# Autodesk Inventor assembly: PBLMK-041-A
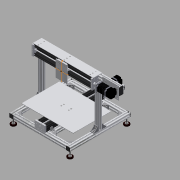
[picture p0: Inventor's stored thumbnail of the model, 180x180]
Saved by Autodesk Inventor 2016 (Build 200138000, 138)
## iProperties
Created: 2023-12-03
Part Number: PBLMK-041-A
Document SubType Name: Assembly
Designer: Riskinova Oktavia
Checked By: RIDWAN
Engr Approved By: RIDWAN
Company: POLITEKNIK NEGERI BATAM
Author: Riskinova Oktavia
Title: MINI CNC ENGRAVER
## Documents named in this file (56)
- D:\PROJECT NOVA 2021-2022\PBLMK-041\NEW KONSEP\PBLMK-041-A.iam
- D:\PROJECT NOVA 2021-2022\PBLMK-041\NEW KONSEP\SKETCH.ipt
- D:\PROJECT NOVA 2021-2022\PBLMK-041\NEW KONSEP\PBLMK-041-A\Frame\Frame0001.iam
- D:\PROJECT NOVA 2021-2022\PBLMK-041\NEW KONSEP\LINEAR ACTUATOR.iam
- D:\PROJECT NOVA 2021-2022\PBLMK-041\PBLMK-041\Solid33.ipt
- D:\PROJECT NOVA 2021-2022\PBLMK-041\PBLMK-041\Solid45.ipt
- D:\PROJECT NOVA 2021-2022\PBLMK-041\PBLMK-041\Solid39.ipt
- D:\PROJECT NOVA 2021-2022\PBLMK-041\PBLMK-041\Solid41.ipt
- D:\PROJECT NOVA 2021-2022\PBLMK-041\PBLMK-041\Solid43.ipt
- D:\PROJECT NOVA 2021-2022\PBLMK-041\PBLMK-041\Solid44.ipt
- D:\PROJECT NOVA 2021-2022\PBLMK-041\PBLMK-041\Solid57.ipt
- D:\PROJECT NOVA 2021-2022\PBLMK-041\PBLMK-041\Solid58.ipt
- D:\PROJECT NOVA 2021-2022\PBLMK-041\PBLMK-041\Solid31.ipt
- D:\PROJECT NOVA 2021-2022\PBLMK-041\PBLMK-041\Solid32.ipt
- D:\PROJECT NOVA 2021-2022\PBLMK-041\PBLMK-041\Solid1.ipt
- D:\PROJECT NOVA 2021-2022\PBLMK-041\PBLMK-041\Solid53.ipt
- D:\PROJECT NOVA 2021-2022\PBLMK-041\PBLMK-041\Solid54.ipt
- D:\PROJECT NOVA 2021-2022\PBLMK-041\PBLMK-041\Solid55.ipt
- D:\PROJECT NOVA 2021-2022\PBLMK-041\PBLMK-041\Solid56.ipt
- D:\PROJECT NOVA 2021-2022\PBLMK-041\PBLMK-041\Solid49.ipt
- D:\PROJECT NOVA 2021-2022\PBLMK-041\PBLMK-041\Solid16.ipt
- D:\PROJECT NOVA 2021-2022\PBLMK-041\PBLMK-041\Solid15.ipt
- D:\PROJECT NOVA 2021-2022\PBLMK-041\PBLMK-041\Solid14.ipt
- D:\PROJECT NOVA 2021-2022\PBLMK-041\PBLMK-041\Solid13.ipt
- D:\PROJECT NOVA 2021-2022\PBLMK-041\PBLMK-041\Solid12.ipt
- D:\PROJECT NOVA 2021-2022\PBLMK-041\PBLMK-041\Solid11.ipt
- D:\PROJECT NOVA 2021-2022\PBLMK-041\PBLMK-041\Solid10.ipt
- D:\PROJECT NOVA 2021-2022\PBLMK-041\PBLMK-041\Solid64.ipt
- D:\PROJECT NOVA 2021-2022\PBLMK-041\PBLMK-041\Solid63.ipt
- D:\PROJECT NOVA 2021-2022\PBLMK-041\PBLMK-041\Solid62.ipt
- D:\PROJECT NOVA 2021-2022\PBLMK-041\PBLMK-041\Solid61.ipt
- D:\PROJECT NOVA 2021-2022\PBLMK-041\PBLMK-041\Solid46.ipt
- D:\PROJECT NOVA 2021-2022\PBLMK-041\PBLMK-041\Solid42.ipt
- D:\PROJECT NOVA 2021-2022\PBLMK-041\PBLMK-041\Solid40.ipt
- D:\PROJECT NOVA 2021-2022\PBLMK-041\PBLMK-041\Solid38.ipt
- D:\PROJECT NOVA 2021-2022\PBLMK-041\PBLMK-041\Solid34.ipt
- D:\PROJECT NOVA 2021-2022\PBLMK-041\NEW KONSEP\BRACKET MOTOR.ipt
- D:\PROJECT NOVA 2021-2022\PBLMK-041\NEW KONSEP\ies23 MOTOR.ipt
- D:\PROJECT NOVA 2021-2022\PBLMK-041\NEW KONSEP\BRACKET MOTOR 2.ipt
- D:\PROJECT NOVA 2021-2022\PBLMK-041\NEW KONSEP\END CAP 30.ipt
- D:\PROJECT NOVA 2021-2022\PBLMK-041\NEW KONSEP\PBLMK-041-1.ipt
- C:\Users\Riskinova Oktavia\Documents\Inventor\Content Center Files\R2016\en-US\ASME ANSI B18.3.5M(2)\ASME_ANSI B18.3.5M - M5x10(2).ipt
- D:\PROJECT NOVA 2021-2022\PBLMK-041\NEW KONSEP\Gusset 30.ipt
- D:\PROJECT NOVA 2021-2022\PBLMK-041\NEW KONSEP\Adjuster Pad.ipt
- D:\PROJECT NOVA 2021-2022\PBLMK-041\NEW KONSEP\PBLMK-041-2.ipt
- C:\Users\Riskinova Oktavia\Documents\Inventor\Content Center Files\R2016\en-US\Cap Screw\Cap - M4 x 16.ipt
- C:\Users\Riskinova Oktavia\Documents\Inventor\Content Center Files\R2016\en-US\ISO 7092\ISO 7092 - ST 4 - 140 HV.ipt
- C:\Users\Riskinova Oktavia\Documents\Inventor\Content Center Files\R2016\en-US\ISO 4036(2)\ISO 4036 - M4(2).ipt
- C:\Users\Riskinova Oktavia\Documents\Inventor\Content Center Files\R2016\en-US\ASME ANSI B18.3.5M(2)\ASME_ANSI B18.3.5M - M5x12(2).ipt
- D:\PROJECT NOVA 2021-2022\PBLMK-041\NEW KONSEP\END CAP 3060.ipt
- C:\Users\Riskinova Oktavia\Documents\Inventor\Content Center Files\R2016\en-US\Cap Screw\Cap - M5 x 12.ipt
- C:\Users\Riskinova Oktavia\Documents\Inventor\Content Center Files\R2016\en-US\Cap Screw\Cap - M5 x 10.ipt
- D:\PROJECT NOVA 2021-2022\PBLMK-041\NEW KONSEP\GUSSET 2020.ipt
- C:\Users\Riskinova Oktavia\Documents\Inventor\Content Center Files\R2016\en-US\ASME ANSI B18.3.5M(2)\ASME_ANSI B18.3.5M - M4x8(2).ipt
- C:\Users\Riskinova Oktavia\Documents\Inventor\Content Center Files\R2016\en-US\Cap Screw\Cap - M3 x 8.ipt
- D:\PROJECT NOVA 2021-2022\PBLMK-041\NEW KONSEP\PBLMK-041-5.ipt
## Components (190 placed, 55 different names)
1. SKETCH:1 — Mate:261, Flush:39
2. Frame0001:1 [sub-assembly] — Mate:96, Flush:6, Mate:107, Mate:214, Flush:34, Mate:232, Mate:274, Mate:275, Flush:37, Mate:277, Flush:38, Mate:280, Flush:40, Mate:295, Mate:296, Mate:297, Mate:298, Flush:42, Mate:300, Mate:301, Mate:302, Flush:43, Mate:303, Mate:304, Mate:305, Flush:45, Mate:306, Mate:307, Mate:308, Mate:309, Mate:310, Mate:311, Mate:312, Flush:49, Mate:313, Flush:50, Mate:314, Mate:315, Mate:316, Flush:51, Mate:317, Mate:318, Mate:319, Mate:320, Mate:321, Flush:54, Flush:55, Mate:453, Flush:57, Flush:58, Mate:458, Mate:467, Mate:468, Mate:469, Mate:470, Mate:475, Mate:476, Mate:477, Mate:478, Mate:479, Mate:480, Mate:481, Mate:482, Mate:483, Mate:484, Mate:489, Mate:490, Mate:526, Mate:527, Mate:528, Mate:529, Mate:536, Flush:68, Flush:69, Mate:537, Flush:70, Flush:71, Flush:72, Mate:538, Flush:73, Flush:74, Mate:539, Flush:75, Flush:76, Mate:540, Mate:541, Mate:542, Mate:543, Mate:544, Mate:545
3. LINEAR ACTUATOR:1 [sub-assembly] — Mate:530, Mate:531, Flush:67, Mate:546, Mate:547
4. Solid33:1 — Mate:105
5. Solid39:1
6. Solid41:1
7. Solid43:1
8. Solid44:1 — Mate:96, Flush:6, Mate:233, Flush:62
9. Solid57:1
10. Solid58:1
11. Solid31:1 — Mate:444, Mate:445, Mate:448
12. Solid1:1 — Mate:446
13. Solid53:1 — Mate:443, Mate:447, Mate:452
14. Solid54:1 — Mate:442, Mate:446, Mate:450, Mate:451
15. Solid55:1 — Mate:443, Mate:444
16. Solid56:1 — Mate:442, Mate:445
17. Solid64:1
18. Solid63:1
19. Solid62:1
20. Solid61:1
21. Solid46:1 — Flush:61
22. Solid42:1
23. Solid40:1
24. Solid38:1
25. Solid34:1 — Mate:109
26. Solid1:2 — Mate:447, Mate:448
27. Solid58:2
28. Solid58:3
29. BRACKET MOTOR:1 — Mate:102, Mate:201, Mate:202, Mate:203, Mate:204, Mate:243, Mate:245, Mate:247, Mate:249
30. ies23 MOTOR:1 — Mate:102, Mate:234, Mate:235, Mate:236, Mate:237, Mate:238, Mate:239, Mate:240, Mate:241
31. ies23 MOTOR:2 — Mate:105, Mate:106, Mate:108, Mate:342, Mate:343, Mate:344, Mate:345, Mate:346, Mate:347, Mate:348, Mate:349, Mate:474
32. BRACKET MOTOR 2:1 — Mate:107, Mate:108, Mate:109, Mate:228, Mate:229, Mate:230, Mate:231, Mate:351, Mate:353, Mate:355, Mate:357, Mate:474
33. END CAP 30:1 — Mate:536, Flush:68, Flush:69
34. END CAP 30:2 — Mate:539, Flush:75, Flush:76
35. END CAP 30:3 — Mate:537, Flush:70, Flush:71, Flush:72
36. END CAP 30:4 — Mate:538, Flush:73, Flush:74
37. PBLMK-041-1:1 — Mate:261, Mate:270, Mate:271, Mate:272, Mate:273, Mate:358, Mate:359, Mate:360
38. Broached Hexagon Socket Flat Countersunk Head Cap Screws - Metric M5x10:1
39. Broached Hexagon Socket Flat Countersunk Head Cap Screws - Metric M5x10:4
40. Broached Hexagon Socket Flat Countersunk Head Cap Screws - Metric M5x10:5 — Mate:201
41. Broached Hexagon Socket Flat Countersunk Head Cap Screws - Metric M5x10:6 — Mate:202
42. Broached Hexagon Socket Flat Countersunk Head Cap Screws - Metric M5x10:7 — Mate:203
43. Broached Hexagon Socket Flat Countersunk Head Cap Screws - Metric M5x10:8 — Mate:204
44. Adjuster Pad:1 — Mate:469, Mate:540
45. Adjuster Pad:2 — Mate:467, Mate:543
46. Adjuster Pad:3 — Mate:470, Mate:541
47. Adjuster Pad:4 — Mate:468, Mate:542
48. PBLMK-041-2:1 — Mate:214, Flush:34, Mate:491, Mate:492, Mate:493, Mate:494, Mate:495, Mate:496, Mate:497, Mate:498, Mate:499
49. Broached Hexagon Socket Flat Countersunk Head Cap Screws - Metric M5x10:9 — Mate:228
50. Broached Hexagon Socket Flat Countersunk Head Cap Screws - Metric M5x10:10 — Mate:229
51. Broached Hexagon Socket Flat Countersunk Head Cap Screws - Metric M5x10:11 — Mate:230
52. Broached Hexagon Socket Flat Countersunk Head Cap Screws - Metric M5x10:12 — Mate:231
53. Solid45:2 — Mate:232, Mate:233, Flush:39, Mate:395, Mate:485, Mate:486, Mate:487, Mate:488
54. Cap Screw M4 x 16:1 — Mate:234, Mate:235, Mate:242, Mate:254
55. Cap Screw M4 x 16:2 — Mate:236, Mate:237, Mate:246, Mate:250
56. Cap Screw M4 x 16:3 — Mate:238, Mate:239, Mate:248, Mate:252
57. Cap Screw M4 x 16:4 — Mate:240, Mate:241, Mate:244, Mate:256
58. ISO 7092 ST 4 - 140 HV:1 — Mate:242, Mate:243, Mate:255
59. ISO 7092 ST 4 - 140 HV:2 — Mate:244, Mate:245, Mate:257
60. ISO 7092 ST 4 - 140 HV:3 — Mate:246, Mate:247, Mate:251
61. ISO 7092 ST 4 - 140 HV:4 — Mate:248, Mate:249, Mate:253
62. ISO 4036 M4:1 — Mate:250, Mate:251
63. ISO 4036 M4:2 — Mate:252, Mate:253
64. ISO 4036 M4:3 — Mate:254, Mate:255
65. ISO 4036 M4:4 — Mate:256, Mate:257
66. Broached Hexagon Socket Flat Countersunk Head Cap Screws - Metric M5x12:1 — Mate:270
67. Broached Hexagon Socket Flat Countersunk Head Cap Screws - Metric M5x12:2 — Mate:271
68. Broached Hexagon Socket Flat Countersunk Head Cap Screws - Metric M5x12:3 — Mate:272
69. Broached Hexagon Socket Flat Countersunk Head Cap Screws - Metric M5x12:4 — Mate:273
70. Gusset 30:7 — Mate:275, Flush:37, Flush:47, Flush:48, Flush:59, Mate:476
71. Gusset 30:8 — Mate:274, Mate:308, Flush:47
72. Gusset 30:10 — Mate:280, Flush:40, Flush:41, Mate:387, Mate:388, Mate:389, Mate:390, Mate:391, Mate:392, Mate:393, Mate:394, Mate:478
73. Gusset 30:11 — Mate:277, Flush:38, Mate:375, Mate:376, Mate:459, Mate:460, Mate:461, Mate:462, Mate:477
74. Gusset 30:12 — Mate:295, Mate:296, Flush:41, Mate:379, Mate:380, Mate:383, Mate:384
75. Gusset 30:13 — Mate:297, Mate:298, Flush:42, Mate:454, Mate:455, Mate:472, Mate:473
76. Gusset 30:14 — Mate:302, Flush:43, Mate:303, Flush:44, Mate:322, Mate:323, Mate:326, Mate:327
77. Gusset 30:15 — Mate:300, Mate:301, Flush:44, Mate:330, Mate:331, Mate:332, Mate:333
78. Gusset 30:17 — Mate:304, Mate:305, Flush:45, Flush:46, Mate:338, Mate:339, Mate:340, Mate:341
79. Gusset 30:18 — Mate:306, Mate:307, Flush:46, Mate:334, Mate:335, Mate:336, Mate:337
80. Gusset 30:19 — Mate:309, Mate:310, Flush:48
81. Gusset 30:20 — Mate:311, Mate:312, Flush:49, Mate:369, Mate:370, Mate:371, Mate:372
82. Gusset 30:21 — Mate:313, Flush:50, Mate:314, Mate:361, Mate:362, Mate:365, Mate:366
83. Gusset 30:22 — Mate:317, Flush:52, Mate:318, Flush:53, Mate:549
84. Gusset 30:23 — Mate:315, Mate:316, Flush:51, Flush:52, Mate:548, Mate:554, Mate:555, Mate:556, Mate:557
85. Gusset 30:24 — Mate:319, Flush:53, Mate:320, Mate:550, Mate:551, Mate:552, Mate:553
86. END CAP 3060:1 — Mate:321, Flush:54, Flush:55
87. Cap Screw M5 x 12:8 — Mate:322, Mate:323
88. Cap Screw M5 x 10:5 — Mate:326, Mate:327
89. Cap Screw M5 x 10:6 — Mate:330, Mate:331
90. Cap Screw M5 x 10:7 — Mate:332, Mate:333
91. Cap Screw M5 x 12:9 — Mate:334, Mate:335
92. Cap Screw M5 x 12:10 — Mate:336, Mate:337
93. Cap Screw M5 x 12:11 — Mate:338, Mate:339
94. Cap Screw M5 x 12:12 — Mate:340, Mate:341
95. Cap Screw M4 x 16:5 — Mate:342, Mate:343, Mate:350
96. Cap Screw M4 x 16:6 — Mate:344, Mate:345, Mate:352
97. Cap Screw M4 x 16:7 — Mate:346, Mate:347, Mate:356
98. Cap Screw M4 x 16:8 — Mate:348, Mate:349, Mate:354
99. ISO 4036 M4:5 — Mate:350, Mate:351
100. ISO 4036 M4:6 — Mate:352, Mate:353
101. ISO 4036 M4:7 — Mate:354, Mate:355
102. ISO 4036 M4:8 — Mate:356, Mate:357
103. Solid32:2 — Mate:358, Mate:359, Mate:360, Mate:395, Mate:432, Mate:433, Mate:434, Mate:435, Mate:436, Mate:437, Mate:438, Mate:439, Mate:440, Mate:441, Mate:450, Mate:451, Mate:452
104. Cap Screw M5 x 12:13 — Mate:361, Mate:362
105. Cap Screw M5 x 12:14 — Mate:365, Mate:366
106. Cap Screw M5 x 12:15 — Mate:369, Mate:370
107. Cap Screw M5 x 12:16 — Mate:371, Mate:372
108. Cap Screw M5 x 12:17 — Mate:375, Mate:376
109. Cap Screw M5 x 12:18 — Mate:379, Mate:380
110. Cap Screw M5 x 12:19 — Mate:383, Mate:384
111. Cap Screw M5 x 12:20 — Mate:387, Mate:388
112. Cap Screw M5 x 12:21 — Mate:389, Mate:390
113. Cap Screw M5 x 12:22 — Mate:391, Mate:392
114. Cap Screw M5 x 12:23 — Mate:393, Mate:394
115. Solid49:5 — Mate:440
116. Solid16:5
117. Solid15:5
118. Solid14:5
119. Solid13:5
120. Solid12:5
121. Solid11:5
122. Solid10:5 — Mate:432
123. Solid49:6 — Mate:441
124. Solid16:6
125. Solid15:6
126. Solid14:6
127. Solid13:6
128. Solid12:6
129. Solid11:6
130. Solid10:6 — Mate:433
131. Solid49:7 — Mate:439
132. Solid16:7
133. Solid15:7
134. Solid14:7
135. Solid13:7
136. Solid12:7
137. Solid11:7
138. Solid10:7 — Mate:435, Mate:437
139. Solid49:8 — Mate:438
140. Solid16:8
141. Solid15:8
142. Solid14:8
143. Solid13:8
144. Solid12:8
145. Solid11:8
146. Solid10:8 — Mate:434, Mate:436
147. END CAP 3060:2 — Mate:453, Flush:57, Flush:58
148. Cap Screw M5 x 12:24 — Mate:454, Mate:455
149. Gusset 30:25 — Mate:458, Flush:59, Mate:475, Flush:60
150. Cap Screw M5 x 12:25 — Mate:459, Mate:460
151. Cap Screw M5 x 12:26 — Mate:461, Mate:462
152. Cap Screw M5 x 12:27 — Mate:472, Mate:473
153. Gusset 30:26 — Mate:479, Mate:480, Flush:60, Flush:65
154. Gusset 30:28 — Mate:481, Mate:482, Flush:66
155. GUSSET 2020:1 — Mate:483, Mate:486, Flush:64, Mate:502, Mate:503, Mate:518, Mate:519
156. GUSSET 2020:2 — Mate:484, Mate:485, Flush:63, Mate:500, Mate:501, Mate:506, Mate:507
157. GUSSET 2020:3 — Mate:487, Mate:489, Flush:61, Flush:64, Mate:516, Mate:517, Mate:520, Mate:521, Mate:522, Mate:523
158. GUSSET 2020:4 — Mate:488, Mate:490, Flush:62, Flush:63, Mate:512, Mate:513, Mate:524, Mate:525
159. Broached Hexagon Socket Flat Countersunk Head Cap Screws - Metric M4x8:1 — Mate:491
160. Broached Hexagon Socket Flat Countersunk Head Cap Screws - Metric M4x8:2 — Mate:492
161. Broached Hexagon Socket Flat Countersunk Head Cap Screws - Metric M4x8:3 — Mate:493
162. Broached Hexagon Socket Flat Countersunk Head Cap Screws - Metric M4x8:4 — Mate:494
163. Broached Hexagon Socket Flat Countersunk Head Cap Screws - Metric M4x8:5 — Mate:495
164. Broached Hexagon Socket Flat Countersunk Head Cap Screws - Metric M4x8:6 — Mate:496
165. Broached Hexagon Socket Flat Countersunk Head Cap Screws - Metric M4x8:7 — Mate:497
166. Broached Hexagon Socket Flat Countersunk Head Cap Screws - Metric M4x8:8 — Mate:498
167. Broached Hexagon Socket Flat Countersunk Head Cap Screws - Metric M4x8:9 — Mate:499
168. Cap Screw M3 x 8:3 — Mate:500, Mate:501
169. Cap Screw M3 x 8:1 — Mate:502, Mate:503
170. Cap Screw M3 x 8:4 — Mate:506, Mate:507
171. Cap Screw M3 x 8:7 — Mate:512, Mate:513
172. Cap Screw M3 x 8:9 — Mate:516, Mate:517
173. Cap Screw M3 x 8:10 — Mate:518, Mate:519
174. Cap Screw M3 x 8:11 — Mate:520, Mate:521
175. Cap Screw M3 x 8:12 — Mate:522, Mate:523
176. Cap Screw M3 x 8:13 — Mate:524, Mate:525
177. Gusset 30:29 — Mate:526, Mate:527, Flush:65
178. Gusset 30:30 — Mate:528, Mate:529, Flush:66
179. PBLMK-041-5:1 — Mate:530, Mate:531, Flush:67, Mate:532, Mate:533, Mate:534, Mate:535
180. Broached Hexagon Socket Flat Countersunk Head Cap Screws - Metric M5x12:5 — Mate:532
181. Broached Hexagon Socket Flat Countersunk Head Cap Screws - Metric M5x12:6 — Mate:533
182. Broached Hexagon Socket Flat Countersunk Head Cap Screws - Metric M5x12:7 — Mate:534
183. Broached Hexagon Socket Flat Countersunk Head Cap Screws - Metric M5x12:8 — Mate:535
184. GUSSET 2020:5 — Mate:545, Mate:546, Mate:549
185. GUSSET 2020:6 — Mate:544, Mate:547, Mate:548
186. Cap Screw M5 x 12:28 — Mate:550, Mate:551
187. Cap Screw M5 x 12:29 — Mate:552, Mate:553
188. Cap Screw M5 x 12:30 — Mate:554, Mate:555
189. Cap Screw M5 x 12:31 — Mate:556, Mate:557
190. Solid45:1 — Mate:106
## Relationships (378: Mate 318, Flush 44, RevoluteJoint 16)
- [Mate]: Solid33:1 ↔ Solid31:1
- [Mate]: Solid31:1 ↔ Solid45:1
- [Mate]: Solid31:1 ↔ Solid56:1
- [Mate]: Solid31:1 ↔ Solid55:1
- [Mate]: Solid31:1 ↔ Solid1:1
- [Mate]: Solid33:1 ↔ Solid46:1
- [Mate]: Solid33:1 ↔ Solid34:1
- [Mate]: Solid46:1 ↔ Solid34:1
- [Flush]: Solid33:1 ↔ Solid34:1
- [Mate]: Solid46:1 ↔ Solid42:1
- [Mate]: Solid33:1 ↔ Solid40:1
- [Mate]: Solid42:1 ↔ Solid40:1
- [Mate]: Solid33:1 ↔ Solid38:1
- [Mate]: Solid40:1 ↔ Solid38:1
- [Mate]: Solid46:1 ↔ Solid45:1
- [Flush]: Solid46:1 ↔ Solid45:1
- [Mate]: Solid33:1 ↔ Solid39:1
- [Mate]: Solid33:1 ↔ Solid43:1
- [Mate]: Solid33:1 ↔ Solid41:1
- [Mate]: Solid39:1 ↔ Solid41:1
- [Mate]: Solid41:1 ↔ Solid43:1
- [Mate]: Solid44:1 ↔ Solid45:1
- [Flush]: Solid44:1 ↔ Solid45:1
- [Mate]: Solid43:1 ↔ Solid44:1
- [Mate]: Solid44:1 ↔ Solid57:1
- [Mate]: Solid44:1 ↔ Solid58:1
- [Mate]: Solid44:1 ↔ Solid57:1
- [Mate]: Solid44:1 ↔ Solid58:1
- [Mate]: Solid61:1 ↔ Solid46:1
- [Mate]: Solid62:1 ↔ Solid46:1
- [Mate]: Solid63:1 ↔ Solid46:1
- [Mate]: Solid64:1 ↔ Solid46:1
- [Mate]: Solid61:1 ↔ Solid46:1
- [Mate]: Solid63:1 ↔ Solid46:1
- [Mate]: Solid64:1 ↔ Solid46:1
- [Mate]: Solid62:1 ↔ Solid46:1
- [Mate]: Solid44:1 ↔ Solid58:2
- [Mate]: Solid44:1 ↔ Solid58:3
- [Mate]: Solid44:1 ↔ Solid58:2
- [Mate]: Solid44:1 ↔ Solid58:3
- Mate:96: Frame0001:1 ↔ Solid44:1
- Flush:6: Frame0001:1 ↔ Solid44:1
- Mate:102: BRACKET MOTOR:1 ↔ ies23 MOTOR:1
- Mate:105: Solid33:1 ↔ ies23 MOTOR:2
- Mate:106: ies23 MOTOR:2 ↔ Solid45:1
- Mate:107: Frame0001:1 ↔ BRACKET MOTOR 2:1
- Mate:108: ies23 MOTOR:2 ↔ BRACKET MOTOR 2:1
- Mate:109 (10 mm): Solid34:1 ↔ BRACKET MOTOR 2:1
- Mate:201: BRACKET MOTOR:1 ↔ Broached Hexagon Socket Flat Countersunk Head Cap Screws - Metric M5x10:5
- Mate:202: BRACKET MOTOR:1 ↔ Broached Hexagon Socket Flat Countersunk Head Cap Screws - Metric M5x10:6
- Mate:203: BRACKET MOTOR:1 ↔ Broached Hexagon Socket Flat Countersunk Head Cap Screws - Metric M5x10:7
- Mate:204: BRACKET MOTOR:1 ↔ Broached Hexagon Socket Flat Countersunk Head Cap Screws - Metric M5x10:8
- Mate:214: Frame0001:1 ↔ PBLMK-041-2:1
- Flush:34: Frame0001:1 ↔ PBLMK-041-2:1
- Mate:228: BRACKET MOTOR 2:1 ↔ Broached Hexagon Socket Flat Countersunk Head Cap Screws - Metric M5x10:9
- Mate:229: BRACKET MOTOR 2:1 ↔ Broached Hexagon Socket Flat Countersunk Head Cap Screws - Metric M5x10:10
- Mate:230: BRACKET MOTOR 2:1 ↔ Broached Hexagon Socket Flat Countersunk Head Cap Screws - Metric M5x10:11
- Mate:231: BRACKET MOTOR 2:1 ↔ Broached Hexagon Socket Flat Countersunk Head Cap Screws - Metric M5x10:12
- Mate:232: Frame0001:1 ↔ Solid45:2
- Mate:233: Solid44:1 ↔ Solid45:2
- Mate:234: ies23 MOTOR:1 ↔ Cap Screw M4 x 16:1
- Mate:235: ies23 MOTOR:1 ↔ Cap Screw M4 x 16:1
- Mate:236: ies23 MOTOR:1 ↔ Cap Screw M4 x 16:2
- Mate:237: ies23 MOTOR:1 ↔ Cap Screw M4 x 16:2
- Mate:238: ies23 MOTOR:1 ↔ Cap Screw M4 x 16:3
- Mate:239: ies23 MOTOR:1 ↔ Cap Screw M4 x 16:3
- Mate:240: ies23 MOTOR:1 ↔ Cap Screw M4 x 16:4
- Mate:241: ies23 MOTOR:1 ↔ Cap Screw M4 x 16:4
- Mate:242: Cap Screw M4 x 16:1 ↔ ISO 7092 ST 4 - 140 HV:1
- Mate:243: BRACKET MOTOR:1 ↔ ISO 7092 ST 4 - 140 HV:1
- Mate:244: Cap Screw M4 x 16:4 ↔ ISO 7092 ST 4 - 140 HV:2
- Mate:245: BRACKET MOTOR:1 ↔ ISO 7092 ST 4 - 140 HV:2
- Mate:246: Cap Screw M4 x 16:2 ↔ ISO 7092 ST 4 - 140 HV:3
- Mate:247: BRACKET MOTOR:1 ↔ ISO 7092 ST 4 - 140 HV:3
- Mate:248: Cap Screw M4 x 16:3 ↔ ISO 7092 ST 4 - 140 HV:4
- Mate:249: BRACKET MOTOR:1 ↔ ISO 7092 ST 4 - 140 HV:4
- Mate:250: Cap Screw M4 x 16:2 ↔ ISO 4036 M4:1
- Mate:251: ISO 7092 ST 4 - 140 HV:3 ↔ ISO 4036 M4:1
- Mate:252: Cap Screw M4 x 16:3 ↔ ISO 4036 M4:2
- Mate:253: ISO 7092 ST 4 - 140 HV:4 ↔ ISO 4036 M4:2
- Mate:254: Cap Screw M4 x 16:1 ↔ ISO 4036 M4:3
- Mate:255: ISO 7092 ST 4 - 140 HV:1 ↔ ISO 4036 M4:3
- Mate:256: Cap Screw M4 x 16:4 ↔ ISO 4036 M4:4
- Mate:257: ISO 7092 ST 4 - 140 HV:2 ↔ ISO 4036 M4:4
- Mate:261: SKETCH:1 ↔ PBLMK-041-1:1
- Mate:270: PBLMK-041-1:1 ↔ Broached Hexagon Socket Flat Countersunk Head Cap Screws - Metric M5x12:1
- Mate:271: PBLMK-041-1:1 ↔ Broached Hexagon Socket Flat Countersunk Head Cap Screws - Metric M5x12:2
- Mate:272: PBLMK-041-1:1 ↔ Broached Hexagon Socket Flat Countersunk Head Cap Screws - Metric M5x12:3
- Mate:273: PBLMK-041-1:1 ↔ Broached Hexagon Socket Flat Countersunk Head Cap Screws - Metric M5x12:4
- Mate:274: Frame0001:1 ↔ Gusset 30:8
- Mate:275: Frame0001:1 ↔ Gusset 30:7
- Flush:37 (0.75 mm): Frame0001:1 ↔ Gusset 30:7
- Mate:277: Frame0001:1 ↔ Gusset 30:11
- Flush:38 (0.75 mm): Frame0001:1 ↔ Gusset 30:11
- Flush:39: SKETCH:1 ↔ Solid45:2
- Mate:280: Frame0001:1 ↔ Gusset 30:10
- Flush:40 (0.75 mm): Frame0001:1 ↔ Gusset 30:10
- Mate:295: Frame0001:1 ↔ Gusset 30:12
- Mate:296: Frame0001:1 ↔ Gusset 30:12
- Flush:41: Gusset 30:10 ↔ Gusset 30:12
- Mate:297: Frame0001:1 ↔ Gusset 30:13
- Mate:298: Frame0001:1 ↔ Gusset 30:13
- Flush:42 (0.75 mm): Frame0001:1 ↔ Gusset 30:13
- Mate:300: Frame0001:1 ↔ Gusset 30:15
- Mate:301: Frame0001:1 ↔ Gusset 30:15
- Mate:302: Frame0001:1 ↔ Gusset 30:14
- Flush:43 (0.75 mm): Frame0001:1 ↔ Gusset 30:14
- Mate:303: Frame0001:1 ↔ Gusset 30:14
- Flush:44: Gusset 30:14 ↔ Gusset 30:15
- Mate:304: Frame0001:1 ↔ Gusset 30:17
- Mate:305: Frame0001:1 ↔ Gusset 30:17
- Flush:45 (0.75 mm): Frame0001:1 ↔ Gusset 30:17
- Mate:306: Frame0001:1 ↔ Gusset 30:18
- Mate:307: Frame0001:1 ↔ Gusset 30:18
- Flush:46: Gusset 30:17 ↔ Gusset 30:18
- Mate:308: Frame0001:1 ↔ Gusset 30:8
- Flush:47: Gusset 30:7 ↔ Gusset 30:8
- Mate:309: Frame0001:1 ↔ Gusset 30:19
- Mate:310: Frame0001:1 ↔ Gusset 30:19
- Flush:48: Gusset 30:7 ↔ Gusset 30:19
- Mate:311: Frame0001:1 ↔ Gusset 30:20
- Mate:312: Frame0001:1 ↔ Gusset 30:20
- Flush:49 (0.75 mm): Frame0001:1 ↔ Gusset 30:20
- Mate:313: Frame0001:1 ↔ Gusset 30:21
- Flush:50 (0.75 mm): Frame0001:1 ↔ Gusset 30:21
- Mate:314: Frame0001:1 ↔ Gusset 30:21
- Mate:315: Frame0001:1 ↔ Gusset 30:23
- Mate:316: Frame0001:1 ↔ Gusset 30:23
- Flush:51 (0.75 mm): Frame0001:1 ↔ Gusset 30:23
- Mate:317: Frame0001:1 ↔ Gusset 30:22
- Flush:52: Gusset 30:22 ↔ Gusset 30:23
- Mate:318: Frame0001:1 ↔ Gusset 30:22
- Mate:319: Frame0001:1 ↔ Gusset 30:24
- Flush:53: Gusset 30:22 ↔ Gusset 30:24
- Mate:320: Frame0001:1 ↔ Gusset 30:24
- Mate:321: Frame0001:1 ↔ END CAP 3060:1
- Flush:54: Frame0001:1 ↔ END CAP 3060:1
- Flush:55: Frame0001:1 ↔ END CAP 3060:1
- Mate:322: Gusset 30:14 ↔ Cap Screw M5 x 12:8
- Mate:323: Gusset 30:14 ↔ Cap Screw M5 x 12:8
- Mate:326: Gusset 30:14 ↔ Cap Screw M5 x 10:5
- Mate:327: Gusset 30:14 ↔ Cap Screw M5 x 10:5
- Mate:330: Gusset 30:15 ↔ Cap Screw M5 x 10:6
- Mate:331: Gusset 30:15 ↔ Cap Screw M5 x 10:6
- Mate:332: Gusset 30:15 ↔ Cap Screw M5 x 10:7
- Mate:333: Gusset 30:15 ↔ Cap Screw M5 x 10:7
- Mate:334: Gusset 30:18 ↔ Cap Screw M5 x 12:9
- Mate:335: Gusset 30:18 ↔ Cap Screw M5 x 12:9
- Mate:336: Gusset 30:18 ↔ Cap Screw M5 x 12:10
- Mate:337: Gusset 30:18 ↔ Cap Screw M5 x 12:10
- Mate:338: Gusset 30:17 ↔ Cap Screw M5 x 12:11
- Mate:339: Gusset 30:17 ↔ Cap Screw M5 x 12:11
- Mate:340: Gusset 30:17 ↔ Cap Screw M5 x 12:12
- Mate:341: Gusset 30:17 ↔ Cap Screw M5 x 12:12
- Mate:342: ies23 MOTOR:2 ↔ Cap Screw M4 x 16:5
- Mate:343: ies23 MOTOR:2 ↔ Cap Screw M4 x 16:5
- Mate:344: ies23 MOTOR:2 ↔ Cap Screw M4 x 16:6
- Mate:345: ies23 MOTOR:2 ↔ Cap Screw M4 x 16:6
- Mate:346: ies23 MOTOR:2 ↔ Cap Screw M4 x 16:7
- Mate:347: ies23 MOTOR:2 ↔ Cap Screw M4 x 16:7
- Mate:348: ies23 MOTOR:2 ↔ Cap Screw M4 x 16:8
- Mate:349: ies23 MOTOR:2 ↔ Cap Screw M4 x 16:8
- Mate:350: Cap Screw M4 x 16:5 ↔ ISO 4036 M4:5
- Mate:351: BRACKET MOTOR 2:1 ↔ ISO 4036 M4:5
- Mate:352: Cap Screw M4 x 16:6 ↔ ISO 4036 M4:6
- Mate:353: BRACKET MOTOR 2:1 ↔ ISO 4036 M4:6
- Mate:354: Cap Screw M4 x 16:8 ↔ ISO 4036 M4:7
- Mate:355: BRACKET MOTOR 2:1 ↔ ISO 4036 M4:7
- Mate:356: Cap Screw M4 x 16:7 ↔ ISO 4036 M4:8
- Mate:357: BRACKET MOTOR 2:1 ↔ ISO 4036 M4:8
- Mate:358: PBLMK-041-1:1 ↔ Solid32:2
- Mate:359: PBLMK-041-1:1 ↔ Solid32:2
- Mate:360: PBLMK-041-1:1 ↔ Solid32:2
- Mate:361: Gusset 30:21 ↔ Cap Screw M5 x 12:13
- Mate:362: Gusset 30:21 ↔ Cap Screw M5 x 12:13
- Mate:365: Gusset 30:21 ↔ Cap Screw M5 x 12:14
- Mate:366: Gusset 30:21 ↔ Cap Screw M5 x 12:14
- Mate:369: Gusset 30:20 ↔ Cap Screw M5 x 12:15
- Mate:370: Gusset 30:20 ↔ Cap Screw M5 x 12:15
- Mate:371: Gusset 30:20 ↔ Cap Screw M5 x 12:16
- Mate:372: Gusset 30:20 ↔ Cap Screw M5 x 12:16
- Mate:375: Gusset 30:11 ↔ Cap Screw M5 x 12:17
- Mate:376: Gusset 30:11 ↔ Cap Screw M5 x 12:17
- Mate:379: Gusset 30:12 ↔ Cap Screw M5 x 12:18
- Mate:380: Gusset 30:12 ↔ Cap Screw M5 x 12:18
- Mate:383: Gusset 30:12 ↔ Cap Screw M5 x 12:19
- Mate:384: Gusset 30:12 ↔ Cap Screw M5 x 12:19
- Mate:387: Gusset 30:10 ↔ Cap Screw M5 x 12:20
- Mate:388: Gusset 30:10 ↔ Cap Screw M5 x 12:20
- Mate:389: Gusset 30:10 ↔ Cap Screw M5 x 12:21
- Mate:390: Gusset 30:10 ↔ Cap Screw M5 x 12:21
- Mate:391: Gusset 30:10 ↔ Cap Screw M5 x 12:22
- Mate:392: Gusset 30:10 ↔ Cap Screw M5 x 12:22
- Mate:393: Gusset 30:10 ↔ Cap Screw M5 x 12:23
- Mate:394: Gusset 30:10 ↔ Cap Screw M5 x 12:23
- Mate:395 (-50 mm): Solid45:2 ↔ Solid32:2
- [RevoluteJoint]: Solid16:5 ↔ Solid14:5
- [Mate]: Solid14:5 ↔ Solid12:5
- [Mate]: Solid14:5 ↔ Solid13:5
- [Mate]: Solid16:5 ↔ Solid11:5
- [RevoluteJoint]: Solid14:5 ↔ Solid13:5
- [Mate]: Solid15:5 ↔ Solid13:5
- [RevoluteJoint]: Solid15:5 ↔ Solid13:5
- [RevoluteJoint]: Solid15:5 ↔ Solid12:5
- [Mate]: Solid12:5 ↔ Solid10:5
- [Mate]: Solid49:5 ↔ Solid15:5
- [Mate]: Solid16:5 ↔ Solid11:5
- [Mate] (2 mm): Solid49:5 ↔ Solid10:5
- [Mate]: Solid12:5 ↔ Solid10:5
- [RevoluteJoint]: Solid16:6 ↔ Solid14:6
- [Mate]: Solid14:6 ↔ Solid12:6
- [Mate]: Solid14:6 ↔ Solid13:6
- [Mate]: Solid16:6 ↔ Solid11:6
- [RevoluteJoint]: Solid14:6 ↔ Solid13:6
- [Mate]: Solid15:6 ↔ Solid13:6
- [RevoluteJoint]: Solid15:6 ↔ Solid13:6
- [RevoluteJoint]: Solid15:6 ↔ Solid12:6
- [Mate]: Solid12:6 ↔ Solid10:6
- [Mate]: Solid49:6 ↔ Solid15:6
- [Mate]: Solid16:6 ↔ Solid11:6
- [Mate] (2 mm): Solid49:6 ↔ Solid10:6
- [Mate]: Solid12:6 ↔ Solid10:6
- [RevoluteJoint]: Solid16:7 ↔ Solid14:7
- [Mate]: Solid14:7 ↔ Solid12:7
- [Mate]: Solid14:7 ↔ Solid13:7
- [Mate]: Solid16:7 ↔ Solid11:7
- [RevoluteJoint]: Solid14:7 ↔ Solid13:7
- [Mate]: Solid15:7 ↔ Solid13:7
- [RevoluteJoint]: Solid15:7 ↔ Solid13:7
- [RevoluteJoint]: Solid15:7 ↔ Solid12:7
- [Mate]: Solid12:7 ↔ Solid10:7
- [Mate]: Solid49:7 ↔ Solid15:7
- [Mate]: Solid16:7 ↔ Solid11:7
- [Mate] (2 mm): Solid49:7 ↔ Solid10:7
- [Mate]: Solid12:7 ↔ Solid10:7
- [RevoluteJoint]: Solid16:8 ↔ Solid14:8
- [Mate]: Solid14:8 ↔ Solid12:8
- [Mate]: Solid14:8 ↔ Solid13:8
- [Mate]: Solid16:8 ↔ Solid11:8
- [RevoluteJoint]: Solid14:8 ↔ Solid13:8
- [Mate]: Solid15:8 ↔ Solid13:8
- [RevoluteJoint]: Solid15:8 ↔ Solid13:8
- [RevoluteJoint]: Solid15:8 ↔ Solid12:8
- [Mate]: Solid12:8 ↔ Solid10:8
- [Mate]: Solid49:8 ↔ Solid15:8
- [Mate]: Solid16:8 ↔ Solid11:8
- [Mate] (2 mm): Solid49:8 ↔ Solid10:8
- [Mate]: Solid12:8 ↔ Solid10:8
- Mate:432: Solid32:2 ↔ Solid10:5
- Mate:433: Solid32:2 ↔ Solid10:6
- Mate:434: Solid32:2 ↔ Solid10:8
- Mate:435: Solid32:2 ↔ Solid10:7
- Mate:436: Solid32:2 ↔ Solid10:8
- Mate:437: Solid32:2 ↔ Solid10:7
- Mate:438: Solid32:2 ↔ Solid49:8
- Mate:439: Solid32:2 ↔ Solid49:7
- Mate:440: Solid32:2 ↔ Solid49:5
- Mate:441: Solid32:2 ↔ Solid49:6
- Mate:442: Solid54:1 ↔ Solid56:1
- Mate:443: Solid53:1 ↔ Solid55:1
- Mate:444: Solid31:1 ↔ Solid55:1
- Mate:445: Solid31:1 ↔ Solid56:1
- Mate:446: Solid1:1 ↔ Solid54:1
- Mate:447: Solid53:1 ↔ Solid1:2
- Mate:448: Solid31:1 ↔ Solid1:2
- Mate:450: Solid54:1 ↔ Solid32:2
- Mate:451: Solid54:1 ↔ Solid32:2
- Mate:452: Solid53:1 ↔ Solid32:2
- Mate:453: Frame0001:1 ↔ END CAP 3060:2
- Flush:57: Frame0001:1 ↔ END CAP 3060:2
- Flush:58: Frame0001:1 ↔ END CAP 3060:2
- Mate:454: Gusset 30:13 ↔ Cap Screw M5 x 12:24
- Mate:455: Gusset 30:13 ↔ Cap Screw M5 x 12:24
- Mate:458: Frame0001:1 ↔ Gusset 30:25
- Flush:59: Gusset 30:7 ↔ Gusset 30:25
- Mate:459: Gusset 30:11 ↔ Cap Screw M5 x 12:25
- Mate:460: Gusset 30:11 ↔ Cap Screw M5 x 12:25
- Mate:461: Gusset 30:11 ↔ Cap Screw M5 x 12:26
- Mate:462: Gusset 30:11 ↔ Cap Screw M5 x 12:26
- Mate:467: Frame0001:1 ↔ Adjuster Pad:2
- Mate:468: Frame0001:1 ↔ Adjuster Pad:4
- Mate:469: Frame0001:1 ↔ Adjuster Pad:1
- Mate:470: Frame0001:1 ↔ Adjuster Pad:3
- Mate:472: Gusset 30:13 ↔ Cap Screw M5 x 12:27
- Mate:473: Gusset 30:13 ↔ Cap Screw M5 x 12:27
- Mate:474: ies23 MOTOR:2 ↔ BRACKET MOTOR 2:1
- Mate:475: Frame0001:1 ↔ Gusset 30:25
- Mate:476: Frame0001:1 ↔ Gusset 30:7
- Mate:477: Frame0001:1 ↔ Gusset 30:11
- Mate:478: Frame0001:1 ↔ Gusset 30:10
- Mate:479: Frame0001:1 ↔ Gusset 30:26
- Mate:480: Frame0001:1 ↔ Gusset 30:26
- Flush:60: Gusset 30:25 ↔ Gusset 30:26
- Mate:481: Frame0001:1 ↔ Gusset 30:28
- Mate:482: Frame0001:1 ↔ Gusset 30:28
- Mate:483: Frame0001:1 ↔ GUSSET 2020:1
- Mate:484: Frame0001:1 ↔ GUSSET 2020:2
- Mate:485: Solid45:2 ↔ GUSSET 2020:2
- Mate:486: Solid45:2 ↔ GUSSET 2020:1
- Mate:487: Solid45:2 ↔ GUSSET 2020:3
- Mate:488: Solid45:2 ↔ GUSSET 2020:4
- Mate:489: Frame0001:1 ↔ GUSSET 2020:3
- Mate:490: Frame0001:1 ↔ GUSSET 2020:4
- Flush:61 (40 mm): Solid46:1 ↔ GUSSET 2020:3
- Flush:62 (-40 mm): Solid44:1 ↔ GUSSET 2020:4
- Flush:63: GUSSET 2020:2 ↔ GUSSET 2020:4
- Flush:64: GUSSET 2020:1 ↔ GUSSET 2020:3
- Mate:491: PBLMK-041-2:1 ↔ Broached Hexagon Socket Flat Countersunk Head Cap Screws - Metric M4x8:1
- Mate:492: PBLMK-041-2:1 ↔ Broached Hexagon Socket Flat Countersunk Head Cap Screws - Metric M4x8:2
- Mate:493: PBLMK-041-2:1 ↔ Broached Hexagon Socket Flat Countersunk Head Cap Screws - Metric M4x8:3
- Mate:494: PBLMK-041-2:1 ↔ Broached Hexagon Socket Flat Countersunk Head Cap Screws - Metric M4x8:4
- Mate:495: PBLMK-041-2:1 ↔ Broached Hexagon Socket Flat Countersunk Head Cap Screws - Metric M4x8:5
- Mate:496: PBLMK-041-2:1 ↔ Broached Hexagon Socket Flat Countersunk Head Cap Screws - Metric M4x8:6
- Mate:497: PBLMK-041-2:1 ↔ Broached Hexagon Socket Flat Countersunk Head Cap Screws - Metric M4x8:7
- Mate:498: PBLMK-041-2:1 ↔ Broached Hexagon Socket Flat Countersunk Head Cap Screws - Metric M4x8:8
- Mate:499: PBLMK-041-2:1 ↔ Broached Hexagon Socket Flat Countersunk Head Cap Screws - Metric M4x8:9
- Mate:500: GUSSET 2020:2 ↔ Cap Screw M3 x 8:3
- Mate:501: GUSSET 2020:2 ↔ Cap Screw M3 x 8:3
- Mate:502: GUSSET 2020:1 ↔ Cap Screw M3 x 8:1
- Mate:503: GUSSET 2020:1 ↔ Cap Screw M3 x 8:1
- Mate:506: GUSSET 2020:2 ↔ Cap Screw M3 x 8:4
- Mate:507: GUSSET 2020:2 ↔ Cap Screw M3 x 8:4
- Mate:512: GUSSET 2020:4 ↔ Cap Screw M3 x 8:7
- Mate:513: GUSSET 2020:4 ↔ Cap Screw M3 x 8:7
- Mate:516: GUSSET 2020:3 ↔ Cap Screw M3 x 8:9
- Mate:517: GUSSET 2020:3 ↔ Cap Screw M3 x 8:9
- Mate:518: GUSSET 2020:1 ↔ Cap Screw M3 x 8:10
- Mate:519: GUSSET 2020:1 ↔ Cap Screw M3 x 8:10
- Mate:520: GUSSET 2020:3 ↔ Cap Screw M3 x 8:11
- Mate:521: GUSSET 2020:3 ↔ Cap Screw M3 x 8:11
- Mate:522: GUSSET 2020:3 ↔ Cap Screw M3 x 8:12
- Mate:523: GUSSET 2020:3 ↔ Cap Screw M3 x 8:12
- Mate:524: GUSSET 2020:4 ↔ Cap Screw M3 x 8:13
- Mate:525: GUSSET 2020:4 ↔ Cap Screw M3 x 8:13
- Mate:526: Frame0001:1 ↔ Gusset 30:29
- Mate:527: Frame0001:1 ↔ Gusset 30:29
- Flush:65: Gusset 30:26 ↔ Gusset 30:29
- Mate:528: Frame0001:1 ↔ Gusset 30:30
- Mate:529: Frame0001:1 ↔ Gusset 30:30
- Flush:66: Gusset 30:28 ↔ Gusset 30:30
- Mate:530: LINEAR ACTUATOR:1 ↔ PBLMK-041-5:1
- Mate:531: LINEAR ACTUATOR:1 ↔ PBLMK-041-5:1
- Flush:67: LINEAR ACTUATOR:1 ↔ PBLMK-041-5:1
- Mate:532: PBLMK-041-5:1 ↔ Broached Hexagon Socket Flat Countersunk Head Cap Screws - Metric M5x12:5
- Mate:533: PBLMK-041-5:1 ↔ Broached Hexagon Socket Flat Countersunk Head Cap Screws - Metric M5x12:6
- Mate:534: PBLMK-041-5:1 ↔ Broached Hexagon Socket Flat Countersunk Head Cap Screws - Metric M5x12:7
- Mate:535: PBLMK-041-5:1 ↔ Broached Hexagon Socket Flat Countersunk Head Cap Screws - Metric M5x12:8
- Mate:536: Frame0001:1 ↔ END CAP 30:1
- Flush:68: Frame0001:1 ↔ END CAP 30:1
- Flush:69: Frame0001:1 ↔ END CAP 30:1
- Mate:537: Frame0001:1 ↔ END CAP 30:3
- Flush:70: Frame0001:1 ↔ END CAP 30:3
- Flush:71: Frame0001:1 ↔ END CAP 30:3
- Flush:72: Frame0001:1 ↔ END CAP 30:3
- Mate:538: Frame0001:1 ↔ END CAP 30:4
- Flush:73: Frame0001:1 ↔ END CAP 30:4
- Flush:74: Frame0001:1 ↔ END CAP 30:4
- Mate:539: Frame0001:1 ↔ END CAP 30:2
- Flush:75: Frame0001:1 ↔ END CAP 30:2
- Flush:76: Frame0001:1 ↔ END CAP 30:2
- Mate:540: Frame0001:1 ↔ Adjuster Pad:1
- Mate:541: Frame0001:1 ↔ Adjuster Pad:3
- Mate:542: Frame0001:1 ↔ Adjuster Pad:4
- Mate:543: Frame0001:1 ↔ Adjuster Pad:2
- Mate:544: Frame0001:1 ↔ GUSSET 2020:6
- Mate:545: Frame0001:1 ↔ GUSSET 2020:5
- Mate:546: LINEAR ACTUATOR:1 ↔ GUSSET 2020:5
- Mate:547: LINEAR ACTUATOR:1 ↔ GUSSET 2020:6
- Mate:548: Gusset 30:23 ↔ GUSSET 2020:6
- Mate:549: Gusset 30:22 ↔ GUSSET 2020:5
- Mate:550: Gusset 30:24 ↔ Cap Screw M5 x 12:28
- Mate:551: Gusset 30:24 ↔ Cap Screw M5 x 12:28
- Mate:552: Gusset 30:24 ↔ Cap Screw M5 x 12:29
- Mate:553: Gusset 30:24 ↔ Cap Screw M5 x 12:29
- Mate:554: Gusset 30:23 ↔ Cap Screw M5 x 12:30
- Mate:555: Gusset 30:23 ↔ Cap Screw M5 x 12:30
- Mate:556: Gusset 30:23 ↔ Cap Screw M5 x 12:31
- Mate:557: Gusset 30:23 ↔ Cap Screw M5 x 12:31
## Named parameters: d47_d129 = 0 mm, d48_d130 = 0 mm, d49_d0 = 0 mm, d243_d1 = 0 mm, d115_d114 = 0 mm, d53_d115 = 0 mm, d54_d116 = 0 mm, d57_d119 = 0 mm, d58_d120 = 0 mm, d61_d123 = 0 mm, d62_d124 = 0 mm, d63_d125 = 0 mm, d64_d126 = 0 mm, d65_d127 = 0 mm, d66_d128 = 0 mm, d67_d103 = 0 mm, d68_d104 = 0 mm, d132_d105 = 0 mm, d133_d106 = 0 mm, d134_d107 = 0 mm, d135_d108 = 0 mm, d73_d109 = 0 mm, d75_d112 = 0 mm, d76_d113 = 0 mm, d142_d93 = 0 mm, d143_d94 = 0 mm, d144_d95 = 0 mm, d82_d96 = 0 mm, d83_d97 = 0 mm, d84_d98 = 0 mm, d85_d99 = 0 mm, d149_d100 = 0 mm, d87_d101 = 0 mm, d151_d102 = 0 mm, d498_d59_d24 = -76.128704 deg, d499_d60_d25 = 0 mm, d500_d61_d26 = 0 mm, d501_d62_d27 = 0 mm, d502_d63_d28 = 2 mm, d503_d47_d29 = 0 mm, d504_d48_d13 = 0 mm, d505_d49_d14 = -9.588935 deg, d506_d50_d15 = 0 mm, d507_d51_d16 = 0 mm, d508_d52_d17 = 0 mm, d509_d53_d18 = 0 mm, d510_d54_d19 = 0.101201 deg, d511_d55_d20 = 0 mm, d512_d56_d21 = 0 mm, d513_d57_d22 = 172.109037 deg, d514_d58_d23 = 0 mm, d515_d59_d24 = -73.846776 deg, d516_d60_d25 = 0 mm, d517_d61_d26 = 0 mm, d518_d62_d27 = 0 mm, d519_d63_d28 = 2 mm, d520_d47_d29 = 0 mm, d521_d48_d13 = 0 mm, d522_d49_d14 = -10.060735 deg, d523_d50_d15 = 0 mm, d524_d51_d16 = 0 mm, d525_d52_d17 = 0 mm, d526_d53_d18 = 0 mm, d527_d54_d19 = 0.097324 deg, d528_d55_d20 = 0 mm, d529_d56_d21 = 0 mm, d530_d57_d22 = 172.097187 deg, d531_d58_d23 = 0 mm, d532_d59_d24 = -73.552651 deg, d533_d60_d25 = 0 mm, d534_d61_d26 = 0 mm, d535_d62_d27 = 0 mm, d536_d63_d28 = 2 mm, d537_d47_d29 = 0 mm, d538_d48_d13 = 0 mm, d539_d49_d14 = -10.054684 deg, d540_d50_d15 = 0 mm, d541_d51_d16 = 0 mm, d542_d52_d17 = 0 mm, d543_d53_d18 = 0 mm, d544_d54_d19 = 0.098965 deg, d545_d55_d20 = 0 mm, d546_d56_d21 = 0 mm, d547_d57_d22 = 172.104711 deg, d548_d58_d23 = 0 mm, d549_d59_d24 = -78.32435 deg, d550_d60_d25 = 0 mm, d551_d61_d26 = 0 mm, d552_d62_d27 = 0 mm, d553_d63_d28 = 2 mm, d554_d47_d29 = 0 mm, d555_d48_d13 = 0 mm, d556_d49_d14 = -9.022238 deg, d557_d50_d15 = 0 mm, d558_d51_d16 = 0 mm, d559_d52_d17 = 0 mm, d560_d53_d18 = 0 mm, d561_d54_d19 = 0.102213 deg, d562_d55_d20 = 0 mm, d563_d56_d21 = 0 mm, d564_d57_d22 = 172.105798 deg, d565_d58_d23 = 0 mm
